# Autodesk Inventor assembly: SoporteServo
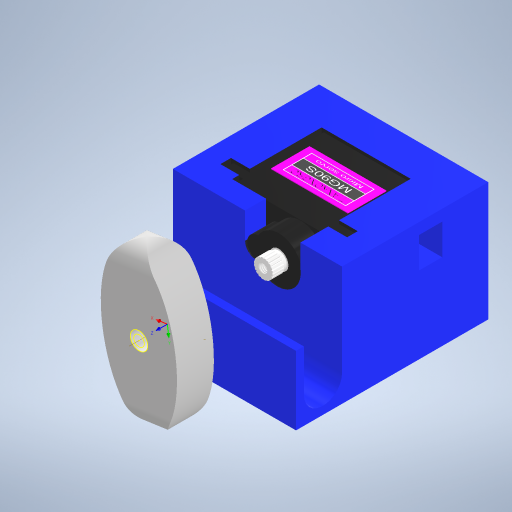
[picture p0: Inventor's stored thumbnail of the model, 512x512]
Saved by Autodesk Inventor 2024.4 (Build 284460000, 460)
## iProperties
Created: 2026-06-02
Part Number: SoporteServo
Document SubType Name: Assembly
Designer: Apleppli
Author: Apleppli
## Documents named in this file (5)
- D:\Downloads\Base_servo\SoporteServo.iam
- D:\Downloads\Base_servo\base.ipt
- D:\Downloads\Base_servo\MG90S\ServoMG90S.iam
- D:\Downloads\Base_servo\bloqueador2XD.ipt
- D:\Downloads\Base_servo\Bidirectional shoulder.ipt
## Components (4 placed, 4 different names)
1. base:1 — Mate:16, Mate:17, Mate:18, Mate:19
2. ServoMG90S:1 [sub-assembly] — Mate:9, Mate:15, Mate:17, Mate:18, Mate:19
3. bloqueador2XD:1 — Mate:9, Mate:12, Mate:13, Mate:14, Mate:15, Mate:16
4. Bidirectional shoulder:1 — Mate:12, Mate:13, Mate:14
## Relationships (9: Mate 9)
- Mate:9: ServoMG90S:1 ↔ bloqueador2XD:1
- Mate:12: bloqueador2XD:1 ↔ Bidirectional shoulder:1
- Mate:13: bloqueador2XD:1 ↔ Bidirectional shoulder:1
- Mate:14: bloqueador2XD:1 ↔ Bidirectional shoulder:1
- Mate:15: ServoMG90S:1 ↔ bloqueador2XD:1
- Mate:16: base:1 ↔ bloqueador2XD:1
- Mate:17: base:1 ↔ ServoMG90S:1
- Mate:18: base:1 ↔ ServoMG90S:1
- Mate:19: base:1 ↔ ServoMG90S:1
